# Autodesk Inventor assembly: ControlHousing
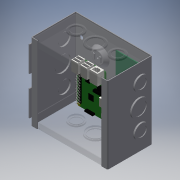
[picture p0: Inventor's stored thumbnail of the model, 180x180]
Saved by Autodesk Inventor 2016 (Build 200138000, 138)
## iProperties
Company: Unknown
Created: 2016-08-11
Part Number: ControlHousing
Description: Unknown
Document SubType Name: Assembly
Designer: jfixelle
Sending System: Unknown
Preprocessor: PSStep 14.0
Title: S:/STOCK/7-COMMERCIAL/CHKO/chko663.stp
Author: Unknown
Revision Number: NONE
## Documents named in this file (8)
- E:\jfixelle\Documents\APC\GitRepo\Control\IAM\ControlHousing.iam
- E:\jfixelle\Downloads\loc13368.ipt
- E:\jfixelle\Downloads\COM55083-4.ipt
- E:\jfixelle\Downloads\COM55563-4.ipt
- E:\jfixelle\Downloads\COM55989.ipt
- E:\jfixelle\Downloads\HNG11000.iam
- E:\jfixelle\Documents\APC\GitRepo\Control\IAM\PiB+.ipt
- E:\jfixelle\Documents\APC\GitRepo\PCB_Libs\3DParts\Prelim_Board.ipt
## Components (9 placed, 9 different names)
1. NAUO4
2. NAUO5
3. NAUO6
4. NAUO7 — Mate:1, Flush:1
5. NAUO8
6. NAUO9 [sub-assembly]
7. NAUO10 [sub-assembly]
8. PiB+:1 — Mate:1
9. Prelim_Board:1 — Flush:1
## Relationships (2: Mate 1, Flush 1)
- Mate:1 (11 mm): NAUO7 ↔ PiB+:1
- Flush:1: NAUO7 ↔ Prelim_Board:1
